# Autodesk Inventor assembly: biggerAct
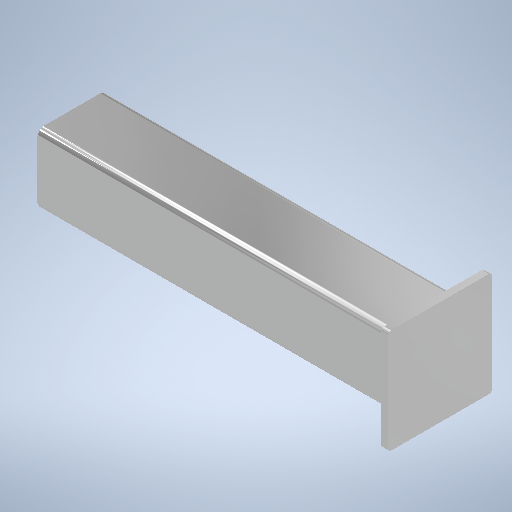
[picture p0: Inventor's stored thumbnail of the model, 512x512]
Saved by Autodesk Inventor 2025.1 (Build 291241000, 241)
## iProperties
Created: 2025-02-26
Part Number: biggerAct
Document SubType Name: Assembly
Designer: yovan
Author: yovan
## Documents named in this file (3)
- C:\Users\yovan\Desktop\APM\ausol-apm.github.io\project\Design and simulation\Inventor\NXModeling\BiggerPneumatic\biggerAct.iam
- C:\Users\yovan\Desktop\APM\ausol-apm.github.io\project\Design and simulation\Inventor\NXModeling\BiggerPneumatic\Contenedor.ipt
- C:\Users\yovan\Desktop\APM\ausol-apm.github.io\project\Design and simulation\Inventor\NXModeling\BiggerPneumatic\Embolo.ipt
## Components (2 placed, 2 different names)
1. Contenedor:1 — Mate:1, Mate:2
2. Embolo:1 — Mate:1, Mate:2
## Relationships (2: Mate 2)
- Mate:1: Contenedor:1 ↔ Embolo:1
- Mate:2 (10 mm): Contenedor:1 ↔ Embolo:1
